# Autodesk Inventor assembly: SDS MK4i Swerve Module, 10-32, NEOs
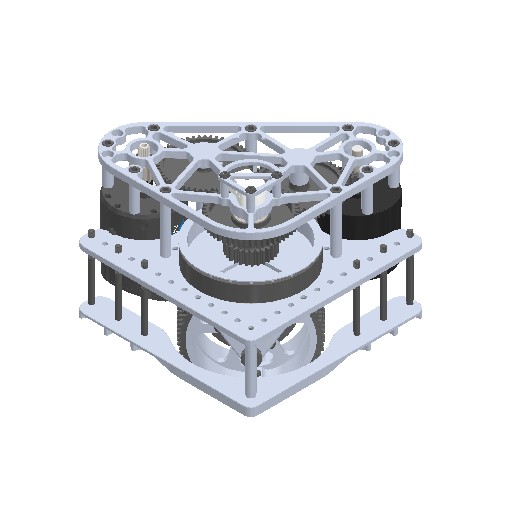
[picture p0: Inventor's stored thumbnail of the model, 512x512]
Saved by Autodesk Inventor 2025.3 (Build 293356000, 356)
## iProperties
Created: 2023-08-16
Part Number: SDS MK4i Swerve Module, 10-32, NEOs
Description: STEP AP214
Document SubType Name: Assembly
Designer: djair.oliveira
Sending System: SolidWorks 2022
Preprocessor: SwSTEP 2.0
Title: SDS MK4i Swerve Module, 10-32, NEOs.STEP
Revision Number: ANY
## Documents named in this file (25)
- C:\Users\djair.oliveira\Desktop\FRC\SEASON 2026\CHASSI DEFAULT\CHASSI\SDS MK4i Swerve Module\SDS MK4i Swerve Module\SDS MK4i Swerve Module, 10-32, NEOs.iam
- C:\Users\djair.oliveira\Desktop\FRC\SEASON 2026\CHASSI DEFAULT\CHASSI\SDS MK4i Swerve Module\SDS MK4i Swerve Module\Screw, 10-32 X .25, Button, 91255A261_91255A261.ipt
- C:\Users\djair.oliveira\Desktop\FRC\SEASON 2026\CHASSI DEFAULT\CHASSI\SDS MK4i Swerve Module\SDS MK4i Swerve Module\Screw, 10-32 X 1.5, 91251A351_91251A351.ipt
- C:\Users\djair.oliveira\Desktop\FRC\SEASON 2026\CHASSI DEFAULT\CHASSI\SDS MK4i Swerve Module\SDS MK4i Swerve Module\Screw, 10-32 X 2.25, 91251A354_91251A354.ipt
- C:\Users\djair.oliveira\Desktop\FRC\SEASON 2026\CHASSI DEFAULT\CHASSI\SDS MK4i Swerve Module\SDS MK4i Swerve Module\Screw, 8-32 X .875, Button, 91255A166_91255A166.ipt
- C:\Users\djair.oliveira\Desktop\FRC\SEASON 2026\CHASSI DEFAULT\CHASSI\SDS MK4i Swerve Module\SDS MK4i Swerve Module\Bearing, 688.ipt
- C:\Users\djair.oliveira\Desktop\FRC\SEASON 2026\CHASSI DEFAULT\CHASSI\SDS MK4i Swerve Module\SDS MK4i Swerve Module\Bearing, R188ZZ.ipt
- C:\Users\djair.oliveira\Desktop\FRC\SEASON 2026\CHASSI DEFAULT\CHASSI\SDS MK4i Swerve Module\SDS MK4i Swerve Module\Gear, 50T, 20DP, .375Hex.ipt
- C:\Users\djair.oliveira\Desktop\FRC\SEASON 2026\CHASSI DEFAULT\CHASSI\SDS MK4i Swerve Module\SDS MK4i Swerve Module\MK4i Steering Shaft Tall.ipt
- C:\Users\djair.oliveira\Desktop\FRC\SEASON 2026\CHASSI DEFAULT\CHASSI\SDS MK4i Swerve Module\SDS MK4i Swerve Module\MK4i Steering Shaft Spacer.ipt
- C:\Users\djair.oliveira\Desktop\FRC\SEASON 2026\CHASSI DEFAULT\CHASSI\SDS MK4i Swerve Module\SDS MK4i Swerve Module\MK4i Shaft, Drive Idler.ipt
- C:\Users\djair.oliveira\Desktop\FRC\SEASON 2026\CHASSI DEFAULT\CHASSI\SDS MK4i Swerve Module\SDS MK4i Swerve Module\Screw, 3-48 X .1875, Pan Phillips, 90272A091_90272A091.ipt
- C:\Users\djair.oliveira\Desktop\FRC\SEASON 2026\CHASSI DEFAULT\CHASSI\SDS MK4i Swerve Module\SDS MK4i Swerve Module\CANcoder Assembly.iam
- C:\Users\djair.oliveira\Desktop\FRC\SEASON 2026\CHASSI DEFAULT\CHASSI\SDS MK4i Swerve Module\SDS MK4i Swerve Module\Motor, NEO.ipt
- C:\Users\djair.oliveira\Desktop\FRC\SEASON 2026\CHASSI DEFAULT\CHASSI\SDS MK4i Swerve Module\SDS MK4i Swerve Module\Shim, 8mm ID X 14mm OD X .5mm Thick, 98055A115_98055A115.ipt
- C:\Users\djair.oliveira\Desktop\FRC\SEASON 2026\CHASSI DEFAULT\CHASSI\SDS MK4i Swerve Module\SDS MK4i Swerve Module\Gear, 20DP, 14T, 8mm REV1.ipt
- C:\Users\djair.oliveira\Desktop\FRC\SEASON 2026\CHASSI DEFAULT\CHASSI\SDS MK4i Swerve Module\SDS MK4i Swerve Module\Retaining Ring, 8mm, 98430A132_98430A132.ipt
- C:\Users\djair.oliveira\Desktop\FRC\SEASON 2026\CHASSI DEFAULT\CHASSI\SDS MK4i Swerve Module\SDS MK4i Swerve Module\Machine Key, 2 X 2 X 12mm.ipt
- C:\Users\djair.oliveira\Desktop\FRC\SEASON 2026\CHASSI DEFAULT\CHASSI\SDS MK4i Swerve Module\SDS MK4i Swerve Module\Belt, 320-5M-15.ipt
- C:\Users\djair.oliveira\Desktop\FRC\SEASON 2026\CHASSI DEFAULT\CHASSI\SDS MK4i Swerve Module\SDS MK4i Swerve Module\MK4 Turret Assembly_Billet Wheel.iam
- C:\Users\djair.oliveira\Desktop\FRC\SEASON 2026\CHASSI DEFAULT\CHASSI\SDS MK4i Swerve Module\SDS MK4i Swerve Module\MK4i Master Part V2_NEO Config.ipt
- C:\Users\djair.oliveira\Desktop\FRC\SEASON 2026\CHASSI DEFAULT\CHASSI\SDS MK4i Swerve Module\SDS MK4i Swerve Module\Screw, 10-32 X 2.5, 91251A355_91251A355.ipt
- C:\Users\djair.oliveira\Desktop\FRC\SEASON 2026\CHASSI DEFAULT\CHASSI\SDS MK4i Swerve Module\SDS MK4i Swerve Module\KRAKEN X60.ipt
- C:\Users\djair.oliveira\Desktop\FRC\SEASON 2026\CHASSI DEFAULT\CHASSI\SDS MK4i Swerve Module\SDS MK4i Swerve Module\Gear, 20DP 14T, Falcon Spline, am-4147.ipt
- C:\Users\djair.oliveira\Desktop\FRC\SEASON 2026\CHASSI DEFAULT\CHASSI\SDS MK4i Swerve Module\Falcon Spacer .25.ipt
## Components (48 placed, 48 different names)
1. Screw, 10-32 X .25, Button, 91255A261_91255A261_1 — Coincidente:30, Alinhado:9
2. Screw, 10-32 X .25, Button, 91255A261_91255A261_2 — Coincidente:36, Coincidente:37
3. Screw, 10-32 X .25, Button, 91255A261_91255A261_3 — Coincidente:32, Alinhado:11, Coincidente:33
4. Screw, 10-32 X .25, Button, 91255A261_91255A261_4 — Coincidente:31, Alinhado:10, Alinhado:11
5. Screw, 10-32 X .25, Button, 91255A261_91255A261_5 — Coincidente:29, Alinhado:9, Alinhado:10
6. Screw, 10-32 X 1.5, 91251A351_91251A351_6 — Coincidente:5, Alinhado:2
7. Screw, 10-32 X 2.25, 91251A354_91251A354_7 — Coincidente:27, Alinhado:8, Coincidente:28
8. Screw, 10-32 X 2.25, 91251A354_91251A354_8 — Coincidente:25, Alinhado:7
9. Screw, 10-32 X 2.25, 91251A354_91251A354_9 — Coincidente:26, Alinhado:7, Alinhado:8
10. Screw, 10-32 X 2.25, 91251A354_91251A354_10 — Coincidente:34, Coincidente:35
11. Screw, 8-32 X .875, Button, 91255A166_91255A166_11 — Alinhado:13, Coincidente:60, Coincidente:61
12. Screw, 8-32 X .875, Button, 91255A166_91255A166_12 — Alinhado:12, Alinhado:13, Coincidente:63
13. Screw, 8-32 X .875, Button, 91255A166_91255A166_13 — Alinhado:12, Coincidente:62
14. Bearing, 688_14 — Coincidente:51, Coincidente:52, Coincidente:58, Coincidente:59
15. Bearing, R188ZZ_15 — Coincidente:44, Coincidente:45, Coincidente:47, Coincidente:48
16. Bearing, 688_16 — Coincidente:40, Coincidente:41
17. Bearing, 688_17 — Coincidente:53, Coincidente:54
18. Gear, 50T, 20DP, .375Hex_18 — Coincidente:55, Coincidente:56, Coincidente:57
19. Gear, 50T, 20DP, .375Hex_19 — Coincidente:38, Coincidente:39, Coincidente:46
20. MK4i Steering Shaft Tall_20 — Coincidente:38, Coincidente:39, Coincidente:42, Coincidente:43, Coincidente:44, Coincidente:45
21. MK4i Steering Shaft Spacer_21 — Coincidente:40, Coincidente:41, Coincidente:42, Coincidente:43, Coincidente:46
22. MK4i Shaft, Drive Idler_22 — Coincidente:51, Coincidente:52, Coincidente:53, Coincidente:54, Coincidente:55, Coincidente:56, Coincidente:57
23. Screw, 3-48 X .1875, Pan Phillips, 90272A091_90272A091_23 — Coincidente:66, Coincidente:68
24. CANcoder Assembly_24 [sub-assembly] — Coincidente:64, Coincidente:65, Coincidente:66, Coincidente:69
25. Screw, 3-48 X .1875, Pan Phillips, 90272A091_90272A091_25 — Coincidente:64, Coincidente:65, Coincidente:67
26. Motor, NEO_27 — Coincidente:1, Coincidente:2, Coincidente:7, Coincidente:22, Coincidente:23, Coincidente:24
27. Shim, 8mm ID X 14mm OD X .5mm Thick, 98055A115_98055A115_28 — Coincidente:18, Coincidente:19, Coincidente:24
28. Gear, 20DP, 14T, 8mm REV1_29 — Coincidente:16, Coincidente:17, Tangente:1, Coincidente:18, Coincidente:19, Coincidente:20, Coincidente:21, Coincidente:22
29. Retaining Ring, 8mm, 98430A132_98430A132_30 — Coincidente:20, Coincidente:21
30. Machine Key, 2 X 2 X 12mm_35 — Coincidente:16, Coincidente:17, Tangente:1, Coincidente:23
31. Belt, 320-5M-15_36 — Coincidente:49, Coincidente:50
32. Screw, 10-32 X 1.5, 91251A351_91251A351_37 — Coincidente:4, Alinhado:1, Alinhado:2, Coincidente:6
33. Screw, 10-32 X 1.5, 91251A351_91251A351_38 — Coincidente:3, Alinhado:1
34. Screw, 10-32 X 1.5, 91251A351_91251A351_39 — Alinhado:14, Coincidente:75, Coincidente:77
35. Screw, 10-32 X 1.5, 91251A351_91251A351_40 — Alinhado:14, Alinhado:15, Coincidente:72, Coincidente:73
36. Screw, 10-32 X 1.5, 91251A351_91251A351_41 — Alinhado:15, Coincidente:74
37. MK4 Turret Assembly_Billet Wheel_42 [sub-assembly] — Coincidente:49, Coincidente:50, Coincidente:70, Coincidente:71
38. MK4i Master Part V2_NEO Config_43 — Coincidente:1, Coincidente:2, Coincidente:3, Coincidente:4, Coincidente:5, Coincidente:6, Coincidente:7, Coincidente:8, Coincidente:9, Coincidente:10, Coincidente:11, Coincidente:12, Coincidente:13, Coincidente:14, Coincidente:15, Coincidente:25, Coincidente:26, Coincidente:27, Coincidente:28, Coincidente:29, Coincidente:30, Coincidente:31, Coincidente:32, Coincidente:33, Coincidente:34, Coincidente:35, Coincidente:36, Coincidente:37, Coincidente:47, Coincidente:48, Coincidente:58, Coincidente:59, Coincidente:60, Coincidente:61, Coincidente:62, Coincidente:63, Coincidente:67, Coincidente:68, Coincidente:69, Coincidente:70, Coincidente:71, Coincidente:72, Coincidente:73, Coincidente:74, Coincidente:75, Coincidente:76, Coincidente:78
39. Screw, 10-32 X 2.5, 91251A355_91251A355_44 — Coincidente:12, Alinhado:5
40. Screw, 10-32 X 2.5, 91251A355_91251A355_45 — Coincidente:13, Alinhado:5, Alinhado:6
41. Screw, 10-32 X 2.5, 91251A355_91251A355_46 — Coincidente:10, Alinhado:3
42. Screw, 10-32 X 2.5, 91251A355_91251A355_47 — Coincidente:9, Alinhado:3, Alinhado:4
43. Screw, 10-32 X 2.5, 91251A355_91251A355_48 — Coincidente:8, Alinhado:4, Coincidente:11
44. Screw, 10-32 X 2.5, 91251A355_91251A355_49 — Coincidente:14, Alinhado:6, Coincidente:15
45. KRAKEN X60:1 — Coincidente:76, Coincidente:77, Coincidente:78, Coincidente:79, Alinhado:16, Coincidente:80, Coincidente:83
46. Gear, 20DP 14T, Falcon Spline, am-4147:1 — Coincidente:79, Alinhado:16, Coincidente:81, Coincidente:82
47. Retaining Ring, 8mm, 98430A132_98430A132:2 — Coincidente:80, Coincidente:81
48. Falcon Spacer .25:1 — Coincidente:82, Coincidente:83
## Relationships (100: Mate 83, Flush 16, Tangent 1)
- Coincidente:1 [Mate]: Motor, NEO_27 ↔ MK4i Master Part V2_NEO Config_43
- Coincidente:2 [Mate]: Motor, NEO_27 ↔ MK4i Master Part V2_NEO Config_43
- Coincidente:3 [Mate]: Screw, 10-32 X 1.5, 91251A351_91251A351_38 ↔ MK4i Master Part V2_NEO Config_43
- Coincidente:4 [Mate]: Screw, 10-32 X 1.5, 91251A351_91251A351_37 ↔ MK4i Master Part V2_NEO Config_43
- Coincidente:5 [Mate]: Screw, 10-32 X 1.5, 91251A351_91251A351_6 ↔ MK4i Master Part V2_NEO Config_43
- Alinhado:1 [Flush]: Screw, 10-32 X 1.5, 91251A351_91251A351_37 ↔ Screw, 10-32 X 1.5, 91251A351_91251A351_38
- Alinhado:2 [Flush]: Screw, 10-32 X 1.5, 91251A351_91251A351_6 ↔ Screw, 10-32 X 1.5, 91251A351_91251A351_37
- Coincidente:6 [Mate]: Screw, 10-32 X 1.5, 91251A351_91251A351_37 ↔ MK4i Master Part V2_NEO Config_43
- Coincidente:7 [Mate]: Motor, NEO_27 ↔ MK4i Master Part V2_NEO Config_43
- Coincidente:8 [Mate]: MK4i Master Part V2_NEO Config_43 ↔ Screw, 10-32 X 2.5, 91251A355_91251A355_48
- Coincidente:9 [Mate]: MK4i Master Part V2_NEO Config_43 ↔ Screw, 10-32 X 2.5, 91251A355_91251A355_47
- Coincidente:10 [Mate]: MK4i Master Part V2_NEO Config_43 ↔ Screw, 10-32 X 2.5, 91251A355_91251A355_46
- Alinhado:3 [Flush]: Screw, 10-32 X 2.5, 91251A355_91251A355_46 ↔ Screw, 10-32 X 2.5, 91251A355_91251A355_47
- Alinhado:4 [Flush]: Screw, 10-32 X 2.5, 91251A355_91251A355_47 ↔ Screw, 10-32 X 2.5, 91251A355_91251A355_48
- Coincidente:11 [Mate]: MK4i Master Part V2_NEO Config_43 ↔ Screw, 10-32 X 2.5, 91251A355_91251A355_48
- Coincidente:12 [Mate]: MK4i Master Part V2_NEO Config_43 ↔ Screw, 10-32 X 2.5, 91251A355_91251A355_44
- Coincidente:13 [Mate]: MK4i Master Part V2_NEO Config_43 ↔ Screw, 10-32 X 2.5, 91251A355_91251A355_45
- Coincidente:14 [Mate]: MK4i Master Part V2_NEO Config_43 ↔ Screw, 10-32 X 2.5, 91251A355_91251A355_49
- Alinhado:5 [Flush]: Screw, 10-32 X 2.5, 91251A355_91251A355_44 ↔ Screw, 10-32 X 2.5, 91251A355_91251A355_45
- Alinhado:6 [Flush]: Screw, 10-32 X 2.5, 91251A355_91251A355_45 ↔ Screw, 10-32 X 2.5, 91251A355_91251A355_49
- Coincidente:15 [Mate]: MK4i Master Part V2_NEO Config_43 ↔ Screw, 10-32 X 2.5, 91251A355_91251A355_49
- Coincidente:16 [Mate]: Gear, 20DP, 14T, 8mm REV1_29 ↔ Machine Key, 2 X 2 X 12mm_35
- Coincidente:17 [Mate]: Gear, 20DP, 14T, 8mm REV1_29 ↔ Machine Key, 2 X 2 X 12mm_35
- Tangente:1: Gear, 20DP, 14T, 8mm REV1_29 ↔ Machine Key, 2 X 2 X 12mm_35
- Coincidente:18 [Mate]: Shim, 8mm ID X 14mm OD X .5mm Thick, 98055A115_98055A115_28 ↔ Gear, 20DP, 14T, 8mm REV1_29
- Coincidente:19 [Mate]: Shim, 8mm ID X 14mm OD X .5mm Thick, 98055A115_98055A115_28 ↔ Gear, 20DP, 14T, 8mm REV1_29
- Coincidente:20 [Mate]: Gear, 20DP, 14T, 8mm REV1_29 ↔ Retaining Ring, 8mm, 98430A132_98430A132_30
- Coincidente:21 [Mate]: Gear, 20DP, 14T, 8mm REV1_29 ↔ Retaining Ring, 8mm, 98430A132_98430A132_30
- Coincidente:22 [Mate]: Motor, NEO_27 ↔ Gear, 20DP, 14T, 8mm REV1_29
- Coincidente:23 [Mate]: Motor, NEO_27 ↔ Machine Key, 2 X 2 X 12mm_35
- Coincidente:24 [Mate]: Motor, NEO_27 ↔ Shim, 8mm ID X 14mm OD X .5mm Thick, 98055A115_98055A115_28
- Coincidente:25 [Mate]: Screw, 10-32 X 2.25, 91251A354_91251A354_8 ↔ MK4i Master Part V2_NEO Config_43
- Coincidente:26 [Mate]: Screw, 10-32 X 2.25, 91251A354_91251A354_9 ↔ MK4i Master Part V2_NEO Config_43
- Coincidente:27 [Mate]: Screw, 10-32 X 2.25, 91251A354_91251A354_7 ↔ MK4i Master Part V2_NEO Config_43
- Alinhado:7 [Flush]: Screw, 10-32 X 2.25, 91251A354_91251A354_8 ↔ Screw, 10-32 X 2.25, 91251A354_91251A354_9
- Alinhado:8 [Flush]: Screw, 10-32 X 2.25, 91251A354_91251A354_7 ↔ Screw, 10-32 X 2.25, 91251A354_91251A354_9
- Coincidente:28 [Mate]: Screw, 10-32 X 2.25, 91251A354_91251A354_7 ↔ MK4i Master Part V2_NEO Config_43
- Coincidente:29 [Mate]: Screw, 10-32 X .25, Button, 91255A261_91255A261_5 ↔ MK4i Master Part V2_NEO Config_43
- Coincidente:30 [Mate]: Screw, 10-32 X .25, Button, 91255A261_91255A261_1 ↔ MK4i Master Part V2_NEO Config_43
- Coincidente:31 [Mate]: Screw, 10-32 X .25, Button, 91255A261_91255A261_4 ↔ MK4i Master Part V2_NEO Config_43
- Coincidente:32 [Mate]: Screw, 10-32 X .25, Button, 91255A261_91255A261_3 ↔ MK4i Master Part V2_NEO Config_43
- Alinhado:9 [Flush]: Screw, 10-32 X .25, Button, 91255A261_91255A261_1 ↔ Screw, 10-32 X .25, Button, 91255A261_91255A261_5
- Alinhado:10 [Flush]: Screw, 10-32 X .25, Button, 91255A261_91255A261_4 ↔ Screw, 10-32 X .25, Button, 91255A261_91255A261_5
- Alinhado:11 [Flush]: Screw, 10-32 X .25, Button, 91255A261_91255A261_3 ↔ Screw, 10-32 X .25, Button, 91255A261_91255A261_4
- Coincidente:33 [Mate]: Screw, 10-32 X .25, Button, 91255A261_91255A261_3 ↔ MK4i Master Part V2_NEO Config_43
- Coincidente:34 [Mate]: Screw, 10-32 X 2.25, 91251A354_91251A354_10 ↔ MK4i Master Part V2_NEO Config_43
- Coincidente:35 [Mate]: Screw, 10-32 X 2.25, 91251A354_91251A354_10 ↔ MK4i Master Part V2_NEO Config_43
- Coincidente:36 [Mate]: Screw, 10-32 X .25, Button, 91255A261_91255A261_2 ↔ MK4i Master Part V2_NEO Config_43
- Coincidente:37 [Mate]: Screw, 10-32 X .25, Button, 91255A261_91255A261_2 ↔ MK4i Master Part V2_NEO Config_43
- Coincidente:38 [Mate]: Gear, 50T, 20DP, .375Hex_19 ↔ MK4i Steering Shaft Tall_20
- Coincidente:39 [Mate]: Gear, 50T, 20DP, .375Hex_19 ↔ MK4i Steering Shaft Tall_20
- Coincidente:40 [Mate]: Bearing, 688_16 ↔ MK4i Steering Shaft Spacer_21
- Coincidente:41 [Mate]: Bearing, 688_16 ↔ MK4i Steering Shaft Spacer_21
- Coincidente:42 [Mate]: MK4i Steering Shaft Tall_20 ↔ MK4i Steering Shaft Spacer_21
- Coincidente:43 [Mate]: MK4i Steering Shaft Tall_20 ↔ MK4i Steering Shaft Spacer_21
- Coincidente:44 [Mate]: Bearing, R188ZZ_15 ↔ MK4i Steering Shaft Tall_20
- Coincidente:45 [Mate]: Bearing, R188ZZ_15 ↔ MK4i Steering Shaft Tall_20
- Coincidente:46 [Mate]: Gear, 50T, 20DP, .375Hex_19 ↔ MK4i Steering Shaft Spacer_21
- Coincidente:47 [Mate]: Bearing, R188ZZ_15 ↔ MK4i Master Part V2_NEO Config_43
- Coincidente:48 [Mate]: Bearing, R188ZZ_15 ↔ MK4i Master Part V2_NEO Config_43
- Coincidente:49 [Mate]: Belt, 320-5M-15_36 ↔ MK4 Turret Assembly_Billet Wheel_42
- Coincidente:50 [Mate] (2 mm): Belt, 320-5M-15_36 ↔ MK4 Turret Assembly_Billet Wheel_42
- Coincidente:51 [Mate]: Bearing, 688_14 ↔ MK4i Shaft, Drive Idler_22
- Coincidente:52 [Mate]: Bearing, 688_14 ↔ MK4i Shaft, Drive Idler_22
- Coincidente:53 [Mate]: Bearing, 688_17 ↔ MK4i Shaft, Drive Idler_22
- Coincidente:54 [Mate]: Bearing, 688_17 ↔ MK4i Shaft, Drive Idler_22
- Coincidente:55 [Mate]: Gear, 50T, 20DP, .375Hex_18 ↔ MK4i Shaft, Drive Idler_22
- Coincidente:56 [Mate]: Gear, 50T, 20DP, .375Hex_18 ↔ MK4i Shaft, Drive Idler_22
- Coincidente:57 [Mate]: Gear, 50T, 20DP, .375Hex_18 ↔ MK4i Shaft, Drive Idler_22
- Coincidente:58 [Mate]: Bearing, 688_14 ↔ MK4i Master Part V2_NEO Config_43
- Coincidente:59 [Mate]: Bearing, 688_14 ↔ MK4i Master Part V2_NEO Config_43
- Alinhado:12 [Flush]: Screw, 8-32 X .875, Button, 91255A166_91255A166_12 ↔ Screw, 8-32 X .875, Button, 91255A166_91255A166_13
- Alinhado:13 [Flush]: Screw, 8-32 X .875, Button, 91255A166_91255A166_11 ↔ Screw, 8-32 X .875, Button, 91255A166_91255A166_12
- Coincidente:60 [Mate]: Screw, 8-32 X .875, Button, 91255A166_91255A166_11 ↔ MK4i Master Part V2_NEO Config_43
- Coincidente:61 [Mate]: Screw, 8-32 X .875, Button, 91255A166_91255A166_11 ↔ MK4i Master Part V2_NEO Config_43
- Coincidente:62 [Mate]: Screw, 8-32 X .875, Button, 91255A166_91255A166_13 ↔ MK4i Master Part V2_NEO Config_43
- Coincidente:63 [Mate]: Screw, 8-32 X .875, Button, 91255A166_91255A166_12 ↔ MK4i Master Part V2_NEO Config_43
- Coincidente:64 [Mate]: CANcoder Assembly_24 ↔ Screw, 3-48 X .1875, Pan Phillips, 90272A091_90272A091_25
- Coincidente:65 [Mate]: CANcoder Assembly_24 ↔ Screw, 3-48 X .1875, Pan Phillips, 90272A091_90272A091_25
- Coincidente:66 [Mate]: Screw, 3-48 X .1875, Pan Phillips, 90272A091_90272A091_23 ↔ CANcoder Assembly_24
- Coincidente:67 [Mate]: Screw, 3-48 X .1875, Pan Phillips, 90272A091_90272A091_25 ↔ MK4i Master Part V2_NEO Config_43
- Coincidente:68 [Mate]: Screw, 3-48 X .1875, Pan Phillips, 90272A091_90272A091_23 ↔ MK4i Master Part V2_NEO Config_43
- Coincidente:69 [Mate]: CANcoder Assembly_24 ↔ MK4i Master Part V2_NEO Config_43
- Coincidente:70 [Mate]: MK4 Turret Assembly_Billet Wheel_42 ↔ MK4i Master Part V2_NEO Config_43
- Coincidente:71 [Mate]: MK4 Turret Assembly_Billet Wheel_42 ↔ MK4i Master Part V2_NEO Config_43
- Alinhado:14 [Flush]: Screw, 10-32 X 1.5, 91251A351_91251A351_39 ↔ Screw, 10-32 X 1.5, 91251A351_91251A351_40
- Alinhado:15 [Flush]: Screw, 10-32 X 1.5, 91251A351_91251A351_40 ↔ Screw, 10-32 X 1.5, 91251A351_91251A351_41
- Coincidente:72 [Mate]: Screw, 10-32 X 1.5, 91251A351_91251A351_40 ↔ MK4i Master Part V2_NEO Config_43
- Coincidente:73 [Mate]: Screw, 10-32 X 1.5, 91251A351_91251A351_40 ↔ MK4i Master Part V2_NEO Config_43
- Coincidente:74 [Mate]: Screw, 10-32 X 1.5, 91251A351_91251A351_41 ↔ MK4i Master Part V2_NEO Config_43
- Coincidente:75 [Mate]: Screw, 10-32 X 1.5, 91251A351_91251A351_39 ↔ MK4i Master Part V2_NEO Config_43
- Coincidente:76 [Mate]: MK4i Master Part V2_NEO Config_43 ↔ KRAKEN X60:1
- Coincidente:77 [Mate]: Screw, 10-32 X 1.5, 91251A351_91251A351_39 ↔ KRAKEN X60:1
- Coincidente:78 [Mate]: MK4i Master Part V2_NEO Config_43 ↔ KRAKEN X60:1
- Coincidente:79 [Mate]: KRAKEN X60:1 ↔ Gear, 20DP 14T, Falcon Spline, am-4147:1
- Alinhado:16 [Flush] (12 mm): KRAKEN X60:1 ↔ Gear, 20DP 14T, Falcon Spline, am-4147:1
- Coincidente:80 [Mate]: KRAKEN X60:1 ↔ Retaining Ring, 8mm, 98430A132_98430A132:2
- Coincidente:81 [Mate]: Gear, 20DP 14T, Falcon Spline, am-4147:1 ↔ Retaining Ring, 8mm, 98430A132_98430A132:2
- Coincidente:82 [Mate]: Gear, 20DP 14T, Falcon Spline, am-4147:1 ↔ Falcon Spacer .25:1
- Coincidente:83 [Mate]: KRAKEN X60:1 ↔ Falcon Spacer .25:1
